# Autodesk Inventor assembly: Assembly1
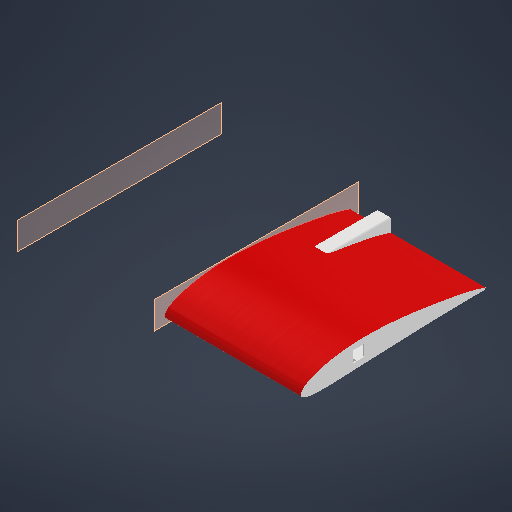
[picture p0: Inventor's stored thumbnail of the model, 512x512]
Saved by Autodesk Inventor 2026.2 (Build 302298010, 298A)
## iProperties
Created: 2026-03-24
Part Number: Assembly1
Document SubType Name: Assembly
Designer: samue
Author: samue
## Documents named in this file (2)
- C:\Users\samue\Documents\GitHub\Senior-Design-UAV\Elytra CAD\Assembly1.iam
- C:\Users\samue\OneDrive - University of South Carolina\Hansen, Madeline's files - Senior Design UAV\Development\Structural Analysis\Modified CAD\V3.0\WingLeft_Junct.ipt
## Components (1 placed, 1 different names)
1. WingLeft_Junct:2 — Flush:1, Flush:3
## Relationships (3: Flush 3)
- Flush:1: WingLeft_Junct:2
- Flush:2 (246.0625 mm)
- Flush:3: WingLeft_Junct:2
